# Autodesk Inventor assembly: total_assembly
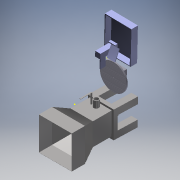
[picture p0: Inventor's stored thumbnail of the model, 180x180]
Saved by Autodesk Inventor 2019 (Build 230136000, 136)
## iProperties
Created: 2020-02-19
Part Number: total_assembly
Document SubType Name: Assembly
Designer: Chirag
Author: Chirag
## Documents named in this file (5)
- E:\Virtual_implementation\zip_ipt_iam\total_assembly.iam
- E:\Virtual_implementation\zip_ipt_iam\helical_screw.ipt
- E:\Virtual_implementation\zip_ipt_iam\This_is_my_deigns.ipt
- E:\Virtual_implementation\zip_ipt_iam\subsystem_4.ipt
- C:\Users\Chirag\Downloads\subsytem-3assembly.iam
## Components (4 placed, 4 different names)
1. helical_screw:1 — Cylindrical:1
2. This_is_my_deigns:1 — Cylindrical:1
3. subsystem_4:1
4. subsytem-3assembly:1 [sub-assembly]
## Relationships (1: CylindricalJoint 1)
- Cylindrical:1: helical_screw:1 ↔ This_is_my_deigns:1
